# Autodesk Inventor assembly: Foot_MIR
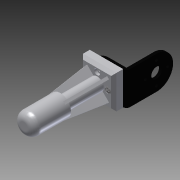
[picture p0: Inventor's stored thumbnail of the model, 180x180]
Saved by Autodesk Inventor 2015 (Build 190159000, 159)
## iProperties
Created: 2015-05-22
Part Number: Foot_MIR
Document SubType Name: Assembly
Designer: Quinn
Author: Quinn
## Documents named in this file (3)
- C:\Users\Quinn\Desktop\3DCNC Design\InventorModels\Assemblies\Foot_MIR.iam
- C:\Users\Quinn\Desktop\3DCNC Design\InventorModels\Plastics\QuadrupedFoot_MIR.ipt
- C:\Users\Quinn\Desktop\3DCNC Design\InventorModels\Metal\Brackets\asb-06-LTab_MIR.ipt
## Components (2 placed, 2 different names)
1. QuadrupedFoot_MIR:1 — Insert:1
2. asb-06-LTab_MIR:1 — Insert:1
## Relationships (1: Insert 1)
- Insert:1: QuadrupedFoot_MIR:1 ↔ asb-06-LTab_MIR:1
